# Autodesk Inventor assembly: Tractor_Plates
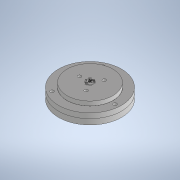
[picture p0: Inventor's stored thumbnail of the model, 180x180]
Saved by Autodesk Inventor 2022 (Build 260153070, 153G)
## iProperties
Created: 2022-03-05
Part Number: Tractor_Plates
Document SubType Name: Assembly
Designer: a laptop
Author: a laptop
## Documents named in this file (9)
- C:\Users\a laptop\Desktop\MDL_2021_Project\Tractor_Plates.iam
- C:\Users\a laptop\Desktop\MDL_2021_Project\Tractor_Static.ipt
- C:\Users\a laptop\Desktop\MDL_2021_Project\Tractor_Mobile.ipt
- C:\Users\a laptop\Desktop\MDL_2021_Project\Tractor_Plates\Design Accelerator\Bearing1.iam
- C:\Users\a laptop\Desktop\MDL_2021_Project\Slip_Ring.ipt
- C:\Users\a laptop\Desktop\MDL_2021_Project\AS5600.ipt
- C:\Users\a laptop\Desktop\MDL_2021_Project\Magnet.ipt
- C:\Users\a laptop\Desktop\MDL_2021_Project\Tractor_Mobile_2.ipt
- C:\Users\a laptop\Desktop\MDL_2021_Project\Tractor_Static_2.ipt
## Components (8 placed, 8 different names)
1. Tractor_Static:1 — Mate:1, Mate:2, Mate:3, Mate:4, Mate:5, Flush:1, Mate:12, Mate:13, Mate:14
2. Tractor_Mobile:1 — Mate:6, Mate:7, Mate:8, Mate:9, Mate:10, Mate:11
3. Bearing:1 [sub-assembly] — Mate:1, Mate:5, Mate:6, Mate:7
4. Slip_Ring:1 — Mate:2, Flush:1
5. AS5600:1 — Mate:4, Mate:15, Mate:16, Mate:17
6. Magnet:1 — Mate:3
7. Tractor_Mobile_2:1 — Mate:8, Mate:9, Mate:10, Mate:11
8. Tractor_Static_2:1 — Mate:12, Mate:13, Mate:14, Mate:15, Mate:16, Mate:17
## Relationships (18: Mate 17, Flush 1)
- Mate:1: Tractor_Static:1 ↔ Bearing:1
- Mate:2: Tractor_Static:1 ↔ Slip_Ring:1
- Mate:3: Tractor_Static:1 ↔ Magnet:1
- Mate:4: Tractor_Static:1 ↔ AS5600:1
- Mate:5: Tractor_Static:1 ↔ Bearing:1
- Flush:1: Tractor_Static:1 ↔ Slip_Ring:1
- Mate:6: Tractor_Mobile:1 ↔ Bearing:1
- Mate:7: Tractor_Mobile:1 ↔ Bearing:1
- Mate:8: Tractor_Mobile:1 ↔ Tractor_Mobile_2:1
- Mate:9: Tractor_Mobile:1 ↔ Tractor_Mobile_2:1
- Mate:10: Tractor_Mobile:1 ↔ Tractor_Mobile_2:1
- Mate:11: Tractor_Mobile:1 ↔ Tractor_Mobile_2:1
- Mate:12: Tractor_Static:1 ↔ Tractor_Static_2:1
- Mate:13: Tractor_Static:1 ↔ Tractor_Static_2:1
- Mate:14: Tractor_Static:1 ↔ Tractor_Static_2:1
- Mate:15: AS5600:1 ↔ Tractor_Static_2:1
- Mate:16: AS5600:1 ↔ Tractor_Static_2:1
- Mate:17: AS5600:1 ↔ Tractor_Static_2:1
